# Autodesk Inventor assembly: полигон етз_MIR
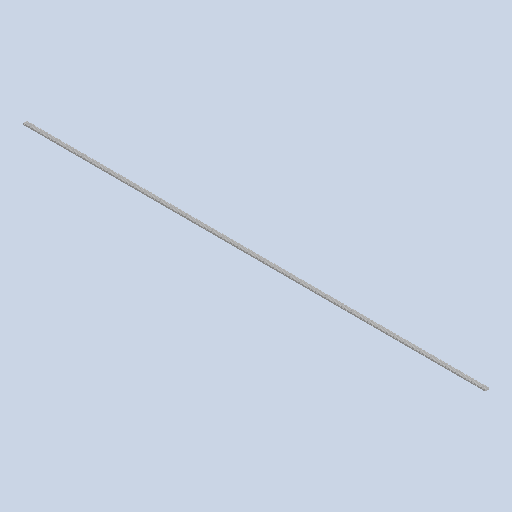
[picture p0: Inventor's stored thumbnail of the model, 512x512]
Saved by Autodesk Inventor 2024.2 (Build 282272000, 272)
## iProperties
Created: 2025-11-16
Part Number: полигон етз_MIR
Document SubType Name: Assembly
Designer: katya_notebook
Author: katya_notebook
## Documents named in this file (2)
- C:\Users\91125\OneDrive\Рабочий стол\alletz\3д модель\полигон\полигон етз_MIR.iam
- C:\Users\91125\OneDrive\Рабочий стол\alletz\3д модель\toothed_rack\m2_20\m2_20_CPY_MIR.ipt
## Components (10 placed, 1 different names)
1. m2_20_CPY_MIR:1 — Совмещение:23, Совмещение:22, Совмещение:21
2. m2_20_CPY_MIR:2 — Совмещение:23, Совмещение:22, Совмещение:21, Совмещение:26, Совмещение:25, Совмещение:24
3. m2_20_CPY_MIR:3 — Совмещение:26, Совмещение:25, Совмещение:24, Совмещение:28, Совмещение:27
4. m2_20_CPY_MIR:4 — Совмещение:28, Совмещение:27, Совмещение:30, Совмещение:29
5. m2_20_CPY_MIR:5 — Совмещение:30, Совмещение:29, Совмещение:34, Совмещение:33
6. m2_20_CPY_MIR:6 — Совмещение:32, Совмещение:31, Совмещение:38, Совмещение:37
7. m2_20_CPY_MIR:7 — Совмещение:32, Совмещение:31, Совмещение:36, Совмещение:35
8. m2_20_CPY_MIR:8 — Совмещение:34, Совмещение:33, Совмещение:40, Совмещение:39
9. m2_20_CPY_MIR:9 — Совмещение:36, Совмещение:35
10. m2_20_CPY_MIR:10 — Совмещение:40, Совмещение:39, Совмещение:38, Совмещение:37
## Relationships (20: Mate 20)
- Совмещение:23 [Mate]: m2_20_CPY_MIR:1 ↔ m2_20_CPY_MIR:2
- Совмещение:22 [Mate]: m2_20_CPY_MIR:1 ↔ m2_20_CPY_MIR:2
- Совмещение:21 [Mate]: m2_20_CPY_MIR:1 ↔ m2_20_CPY_MIR:2
- Совмещение:26 [Mate]: m2_20_CPY_MIR:2 ↔ m2_20_CPY_MIR:3
- Совмещение:25 [Mate]: m2_20_CPY_MIR:2 ↔ m2_20_CPY_MIR:3
- Совмещение:24 [Mate]: m2_20_CPY_MIR:2 ↔ m2_20_CPY_MIR:3
- Совмещение:28 [Mate]: m2_20_CPY_MIR:3 ↔ m2_20_CPY_MIR:4
- Совмещение:27 [Mate]: m2_20_CPY_MIR:3 ↔ m2_20_CPY_MIR:4
- Совмещение:30 [Mate]: m2_20_CPY_MIR:4 ↔ m2_20_CPY_MIR:5
- Совмещение:29 [Mate]: m2_20_CPY_MIR:4 ↔ m2_20_CPY_MIR:5
- Совмещение:32 [Mate]: m2_20_CPY_MIR:6 ↔ m2_20_CPY_MIR:7
- Совмещение:31 [Mate]: m2_20_CPY_MIR:6 ↔ m2_20_CPY_MIR:7
- Совмещение:34 [Mate]: m2_20_CPY_MIR:5 ↔ m2_20_CPY_MIR:8
- Совмещение:33 [Mate]: m2_20_CPY_MIR:5 ↔ m2_20_CPY_MIR:8
- Совмещение:36 [Mate]: m2_20_CPY_MIR:7 ↔ m2_20_CPY_MIR:9
- Совмещение:35 [Mate]: m2_20_CPY_MIR:7 ↔ m2_20_CPY_MIR:9
- Совмещение:40 [Mate]: m2_20_CPY_MIR:8 ↔ m2_20_CPY_MIR:10
- Совмещение:39 [Mate]: m2_20_CPY_MIR:8 ↔ m2_20_CPY_MIR:10
- Совмещение:38 [Mate]: m2_20_CPY_MIR:6 ↔ m2_20_CPY_MIR:10
- Совмещение:37 [Mate]: m2_20_CPY_MIR:6 ↔ m2_20_CPY_MIR:10
